# Autodesk Inventor assembly: Left Claw
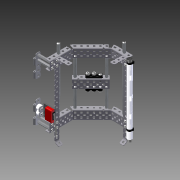
[picture p0: Inventor's stored thumbnail of the model, 180x180]
Saved by Autodesk Inventor 2012 (Build 160160000, 160)
## iProperties
Created: 2011-08-16
Part Number: Left Claw
Document SubType Name: Assembly
Designer: Dakota.Bayer
Author: Dakota.Bayer
## Documents named in this file (26)
- C:\Users\Wade\Documents\1103 Robot - CAD Assembly\Left Claw.iam
- C:\Users\Wade\Documents\1103 Robot - CAD Assembly\2 x 15 bentttttttt.ipt
- C:\Users\Wade\Documents\1103 Robot - CAD Assembly\1 x 20 BENT.ipt
- C:\Users\Wade\Documents\1103 Robot - CAD Assembly\2 x 6 legit.ipt
- C:\Users\Wade\Documents\24C VEX CAD Files\Washers & Spacers\Spacer (Nylon), 0.500''.ipt
- C:\Users\Wade\Documents\24C VEX CAD Files\Standoffs & Couplers\Standoff 2.00''.ipt
- C:\Users\Wade\Documents\24C VEX CAD Files\Other Parts\Shaft Collar (with Set Screw Installed).ipt
- C:\Users\Wade\Documents\24C VEX CAD Files\Other Parts\(Pillow) Bearing Block mod.ipt
- C:\Users\Wade\Documents\24C VEX CAD Files\Washers & Spacers\Spacer (Nylon), 0.250''.ipt
- C:\Users\Wade\Documents\24C VEX CAD Files\Drive Shafts\Drive Shaft (Square Bar) 8''.ipt
- C:\Users\Wade\Documents\1103 Robot - CAD Assembly\VEX-HINGE-2 RevA_1.ipt
- C:\Users\Wade\Documents\1103 Robot - CAD Assembly\Bearing Assembly (end hole).iam
- C:\Users\Wade\Documents\24C VEX CAD Files\Washers & Spacers\Spacer (Nylon), 0.125''.ipt
- C:\Users\Wade\Documents\1103 Robot - CAD Assembly\.375'' Screw & Nylock Nut.iam
- C:\Users\Wade\Documents\24C VEX CAD Files\Standoffs & Couplers\Standoff 5.00''.ipt
- C:\Users\Wade\Documents\24C VEX CAD Files\Screws & Nuts\Screw 8-32 x 0.250''-Silver.ipt
- C:\Users\Wade\Documents\24C VEX CAD Files\Standoffs & Couplers\Standoff 1.50''.ipt
- C:\Users\Wade\Documents\24C VEX CAD Files\Screws & Nuts\Nut 8-32 Nylock.ipt
- C:\Users\Wade\Documents\24C VEX CAD Files\Screws & Nuts\Screw 8-32 x 0.500''-Silver.ipt
- C:\Users\Wade\Documents\24C VEX CAD Files\Standoffs & Couplers\Standoff 1.00''.ipt
- C:\Users\Wade\Documents\24C VEX CAD Files\Motors & Sensors\Limit Switch (Sensor).iam
- C:\Users\Wade\Documents\24C VEX CAD Files\Metal Angles\Short Slotted Angle (Segmented Angle, 1x1x2).ipt
- C:\Users\Wade\Documents\24C VEX CAD Files\Washers & Spacers\Spacer (Nylon), 0.375''.ipt
- C:\Users\Wade\Documents\24C VEX CAD Files\Screws & Nuts\Screw 8-32 x 0.625''-Silver.ipt
- C:\Users\Wade\Documents\24C VEX CAD Files\Washers & Spacers\Spacer (Thin), 4.6mm.ipt
- C:\Users\Wade\Documents\24C VEX CAD Files\Screws & Nuts\Screw 8-32 x 1.750''-Silver.ipt
## Components (93 placed, 25 different names)
1. Standoff 1.50'':1 — Mate:870
2. Standoff 1.50'':2 — Mate:871
3. 2 x 15 bentttttttt:3 — Mate:722, Flush:49, Flush:50, Flush:51, Flush:52, Mate:794, Mate:803, Flush:55, Flush:56, Mate:855, Mate:862, Mate:863, Mate:864, Mate:865, Mate:872, Mate:873, Mate:894, Mate:901, Mate:902, Mate:910, Mate:913, Mate:919, Mate:921
4. Standoff 1.50'':3 — Mate:888, Mate:890
5. Standoff 1.50'':4 — Mate:886, Mate:891
6. 2 x 15 bentttttttt:4 — Mate:796, Mate:797, Mate:804, Mate:805, Mate:806, Flush:57, Mate:851, Mate:879, Mate:881, Mate:883, Mate:885, Mate:892, Mate:893
7. 1 x 20 BENT:3 — Flush:51, Flush:52, Mate:794, Mate:796, Mate:846, Mate:847, Mate:848, Mate:849, Mate:850, Mate:852, Mate:853, Mate:854, Mate:856, Mate:857, Mate:936
8. Standoff 5.00'':1 — Mate:861, Mate:884
9. 2 x 6 legit:2 — Mate:826, Mate:827, Mate:828, Mate:829, Mate:830, Mate:834, Mate:836, Mate:876, Mate:877, Mate:907, Mate:909
10. Standoff 5.00'':2 — Mate:858, Mate:882
11. 1 x 20 BENT:4 — Mate:722, Flush:49, Flush:50, Mate:797, Mate:837, Mate:838, Mate:839, Mate:840, Mate:841, Mate:842, Mate:896, Mate:903
12. Shaft Collar (with Set Screw Installed):1 — Flush:53, Angle:2, Flush:54, Mate:900
13. Shaft Collar (with Set Screw Installed):2 — Mate:815, Flush:54, Flush:58
14. Spacer (Nylon), 0.250'':1 — Mate:808, Mate:809, Mate:810, Mate:811
15. Spacer (Nylon), 0.500'':1 — Mate:808, Mate:809
16. Spacer (Nylon), 0.500'':2 — Mate:810, Mate:811
17. Spacer (Nylon), 0.500'':3
18. Spacer (Nylon), 0.500'':4 — Mate:798, Mate:812, Mate:817
19. Spacer (Nylon), 0.500'':5
20. Spacer (Nylon), 0.500'':6
21. Spacer (Nylon), 0.500'':7
22. Spacer (Nylon), 0.500'':8
23. Spacer (Nylon), 0.500'':9
24. Spacer (Nylon), 0.500'':10
25. Spacer (Nylon), 0.500'':11
26. Spacer (Nylon), 0.500'':12
27. Spacer (Nylon), 0.500'':13 — Mate:798, Mate:813, Mate:814, Mate:815, Mate:818
28. Standoff 2.00'':1 — Mate:859, Mate:874
29. Standoff 2.00'':2 — Mate:860, Mate:875
30. Standoff 2.00'':3 — Mate:880, Mate:906
31. Standoff 2.00'':4 — Mate:878, Mate:908
32. (Pillow) Bearing Block mod:1 — Mate:803, Mate:894, Mate:899, Mate:900, Mate:901, Mate:905
33. (Pillow) Bearing Block mod:2 — Mate:804, Mate:805, Mate:806, Mate:812, Mate:816, Mate:817, Mate:895, Mate:898
34. Spacer (Nylon), 0.250'':2 — Mate:813, Mate:814, Mate:816
35. Drive Shaft (Square Bar) 8'':1 — Mate:818, Flush:53, Angle:2, Flush:58
36. VEX-HINGE-2 RevA_1:1 — Flush:55, Flush:56, Mate:825, Mate:868, Mate:869
37. VEX-HINGE-2 RevA_1:2 — Mate:825, Flush:57, Mate:887, Mate:889, Mate:926, Mate:927, Mate:928, Mate:929, Mate:943, Mate:944
38. Bearing Assembly (end hole):1 [sub-assembly] — Mate:826, Mate:827, Mate:828, Mate:829, Mate:831, Mate:832, Mate:833, Mate:953, Mate:955
39. Bearing Assembly (end hole):2 [sub-assembly] — Mate:830, Mate:831, Mate:832, Mate:835, Mate:956
40. Spacer (Nylon), 0.125'':1 — Mate:833, Mate:834
41. Spacer (Nylon), 0.125'':2 — Mate:835, Mate:836
42. .375'' Screw & Nylock Nut:1 [sub-assembly] — Mate:837, Mate:838, Mate:839
43. .375'' Screw & Nylock Nut:5 [sub-assembly] — Mate:853, Mate:856, Mate:857
44. .375'' Screw & Nylock Nut:7 [sub-assembly] — Mate:840, Mate:841, Mate:842
45. .375'' Screw & Nylock Nut:9 [sub-assembly] — Mate:846, Mate:850, Mate:851
46. .375'' Screw & Nylock Nut:10 [sub-assembly] — Mate:847, Mate:848, Mate:849
47. .375'' Screw & Nylock Nut:12 [sub-assembly] — Mate:852, Mate:854, Mate:855
48. Screw 8-32 x 0.250''-Silver:1 — Mate:859, Mate:864
49. Screw 8-32 x 0.250''-Silver:2 — Mate:858, Mate:865, Mate:911
50. Screw 8-32 x 0.250''-Silver:3 — Mate:860, Mate:863
51. Screw 8-32 x 0.250''-Silver:4 — Mate:861, Mate:862, Mate:912
52. Screw 8-32 x 0.250''-Silver:5 — Mate:868
53. Screw 8-32 x 0.250''-Silver:6 — Mate:869
54. Screw 8-32 x 0.250''-Silver:7 — Mate:870, Mate:872
55. Screw 8-32 x 0.250''-Silver:8 — Mate:871, Mate:873
56. Screw 8-32 x 0.250''-Silver:9 — Mate:875, Mate:877
57. Screw 8-32 x 0.250''-Silver:10 — Mate:874, Mate:876
58. Screw 8-32 x 0.250''-Silver:11 — Mate:880, Mate:881
59. Screw 8-32 x 0.250''-Silver:12 — Mate:878, Mate:879
60. Screw 8-32 x 0.250''-Silver:13 — Mate:882, Mate:883
61. Screw 8-32 x 0.250''-Silver:14 — Mate:884, Mate:885
62. Screw 8-32 x 0.250''-Silver:15 — Mate:888, Mate:889
63. Screw 8-32 x 0.250''-Silver:16 — Mate:886, Mate:887
64. Screw 8-32 x 0.250''-Silver:17 — Mate:891, Mate:893
65. Screw 8-32 x 0.250''-Silver:18 — Mate:890, Mate:892
66. Nut 8-32 Nylock:1 — Mate:897, Mate:898
67. Screw 8-32 x 0.500''-Silver:1 — Mate:895, Mate:896, Mate:897
68. Nut 8-32 Nylock:2 — Mate:904, Mate:905
69. Screw 8-32 x 0.500''-Silver:2 — Mate:899, Mate:902, Mate:903, Mate:904
70. Screw 8-32 x 0.250''-Silver:19 — Mate:906, Mate:907
71. Screw 8-32 x 0.250''-Silver:20 — Mate:908, Mate:909
72. Standoff 1.00'':1 — Mate:910, Mate:911, Mate:914, Mate:915, Mate:920
73. Standoff 1.00'':2 — Mate:912, Mate:913, Mate:916, Mate:917, Mate:918
74. Screw 8-32 x 0.250''-Silver:21 — Mate:914, Mate:915
75. Screw 8-32 x 0.250''-Silver:22 — Mate:916, Mate:917
76. Screw 8-32 x 0.250''-Silver:23 — Mate:920, Mate:921
77. Screw 8-32 x 0.250''-Silver:24 — Mate:918, Mate:919
78. Limit Switch (Sensor):1 [sub-assembly] — Mate:935, Mate:936, Mate:947, Mate:948
79. Screw 8-32 x 0.625''-Silver:3
80. Short Slotted Angle (Segmented Angle, 1x1x2):1 — Mate:922, Mate:923, Mate:924, Mate:925, Mate:932, Mate:933, Mate:934, Mate:939, Mate:951, Mate:952
81. Spacer (Nylon), 0.375'':1 — Mate:922, Mate:924, Mate:926, Mate:929, Mate:937
82. Spacer (Nylon), 0.375'':2 — Mate:923, Mate:925, Mate:927, Mate:928
83. Nut 8-32 Nylock:3 — Mate:950, Mate:951
84. Nut 8-32 Nylock:4 — Mate:942, Mate:944
85. Nut 8-32 Nylock:5 — Mate:943
86. Spacer (Thin), 4.6mm:2 — Mate:934, Mate:945
87. Spacer (Thin), 4.6mm:1 — Mate:932, Mate:933, Mate:935, Mate:946
88. Screw 8-32 x 0.625''-Silver:2 — Mate:937, Mate:939, Mate:942
89. Nut 8-32 Nylock:6 — Mate:949, Mate:952
90. Screw 8-32 x 0.500''-Silver:3 — Mate:946, Mate:948, Mate:949
91. Screw 8-32 x 0.500''-Silver:4 — Mate:945, Mate:947, Mate:950
92. Nut 8-32 Nylock:7 — Mate:954, Mate:956
93. Screw 8-32 x 1.750''-Silver:1 — Mate:953, Mate:954, Mate:955
## Relationships (217: Mate 188, Tangent 18, Flush 10, Angle 1)
- [Mate]: Standoff 1.50'':1 ↔ 2 x 15 bentttttttt:3
- [Tangent] (0.2286 mm): Standoff 1.50'':1 ↔ 2 x 15 bentttttttt:3
- [Tangent] (0.2286 mm): Standoff 1.50'':1 ↔ 2 x 15 bentttttttt:3
- [Tangent] (0.2286 mm): Standoff 1.50'':2 ↔ 2 x 15 bentttttttt:3
- [Mate]: Standoff 1.50'':3 ↔ 2 x 15 bentttttttt:4
- [Tangent] (0.2286 mm): Standoff 1.50'':4 ↔ 2 x 15 bentttttttt:4
- [Tangent] (0.2286 mm): Standoff 1.50'':4 ↔ 2 x 15 bentttttttt:4
- [Tangent] (0.2286 mm): Standoff 1.50'':3 ↔ 2 x 15 bentttttttt:4
- [Mate]: 2 x 15 bentttttttt:3 ↔ Standoff 5.00'':1
- [Tangent] (0.2286 mm): 2 x 15 bentttttttt:3 ↔ Standoff 5.00'':1
- [Tangent] (0.2286 mm): 2 x 15 bentttttttt:3 ↔ Standoff 5.00'':1
- [Mate]: 2 x 15 bentttttttt:3 ↔ Standoff 5.00'':2
- [Tangent] (0.2286 mm): 2 x 15 bentttttttt:3 ↔ Standoff 5.00'':2
- [Tangent] (0.2286 mm): 2 x 15 bentttttttt:3 ↔ Standoff 5.00'':2
- Mate:722: 2 x 15 bentttttttt:3 ↔ 1 x 20 BENT:4
- Flush:49: 2 x 15 bentttttttt:3 ↔ 1 x 20 BENT:4
- Flush:50: 2 x 15 bentttttttt:3 ↔ 1 x 20 BENT:4
- [Mate]: Spacer (Nylon), 0.500'':2 ↔ Spacer (Nylon), 0.500'':3
- [Mate]: Spacer (Nylon), 0.500'':3 ↔ Spacer (Nylon), 0.500'':4
- [Mate]: Spacer (Nylon), 0.500'':2 ↔ Spacer (Nylon), 0.500'':3
- [Mate]: Spacer (Nylon), 0.500'':3 ↔ Spacer (Nylon), 0.500'':4
- [Mate]: Spacer (Nylon), 0.500'':5 ↔ Spacer (Nylon), 0.500'':6
- [Mate]: Spacer (Nylon), 0.500'':5 ↔ Spacer (Nylon), 0.500'':7
- [Mate]: Spacer (Nylon), 0.500'':7 ↔ Spacer (Nylon), 0.500'':8
- [Mate]: Spacer (Nylon), 0.500'':8 ↔ Spacer (Nylon), 0.500'':9
- [Mate]: Spacer (Nylon), 0.500'':9 ↔ Spacer (Nylon), 0.500'':10
- [Mate]: Spacer (Nylon), 0.500'':10 ↔ Spacer (Nylon), 0.500'':11
- [Mate]: Spacer (Nylon), 0.500'':11 ↔ Spacer (Nylon), 0.500'':12
- [Mate]: Spacer (Nylon), 0.500'':5 ↔ Spacer (Nylon), 0.500'':6
- [Mate]: Spacer (Nylon), 0.500'':5 ↔ Spacer (Nylon), 0.500'':7
- [Mate]: Spacer (Nylon), 0.500'':7 ↔ Spacer (Nylon), 0.500'':8
- [Mate]: Spacer (Nylon), 0.500'':8 ↔ Spacer (Nylon), 0.500'':9
- [Mate]: Spacer (Nylon), 0.500'':9 ↔ Spacer (Nylon), 0.500'':10
- [Mate]: Spacer (Nylon), 0.500'':10 ↔ Spacer (Nylon), 0.500'':11
- [Mate]: Spacer (Nylon), 0.500'':11 ↔ Spacer (Nylon), 0.500'':12
- [Mate]: Spacer (Nylon), 0.500'':1 ↔ Spacer (Nylon), 0.500'':12
- [Mate]: Spacer (Nylon), 0.500'':1 ↔ Spacer (Nylon), 0.500'':12
- Flush:51: 2 x 15 bentttttttt:3 ↔ 1 x 20 BENT:3
- Flush:52: 2 x 15 bentttttttt:3 ↔ 1 x 20 BENT:3
- [Mate]: 2 x 6 legit:2 ↔ Standoff 2.00'':1
- [Mate]: 2 x 6 legit:2 ↔ Standoff 2.00'':2
- [Tangent] (0.2286 mm): 2 x 6 legit:2 ↔ Standoff 2.00'':1
- [Tangent] (0.2286 mm): 2 x 6 legit:2 ↔ Standoff 2.00'':1
- [Tangent] (0.2286 mm): 2 x 6 legit:2 ↔ Standoff 2.00'':2
- [Tangent] (0.2286 mm): 2 x 6 legit:2 ↔ Standoff 2.00'':2
- [Mate]: 2 x 15 bentttttttt:3 ↔ Standoff 2.00'':1
- [Tangent] (0.2286 mm): 2 x 15 bentttttttt:3 ↔ Standoff 2.00'':1
- [Tangent] (0.2286 mm): 2 x 15 bentttttttt:3 ↔ Standoff 2.00'':1
- [Tangent] (0.2286 mm): 2 x 15 bentttttttt:3 ↔ Standoff 2.00'':2
- [Tangent] (0.2286 mm): 2 x 15 bentttttttt:3 ↔ Standoff 2.00'':2
- [Mate]: 2 x 6 legit:2 ↔ Standoff 2.00'':3
- [Mate]: 2 x 6 legit:2 ↔ Standoff 2.00'':4
- [Mate]: Standoff 2.00'':2 ↔ Standoff 2.00'':4
- [Mate]: Standoff 2.00'':1 ↔ Standoff 2.00'':3
- Mate:794: 2 x 15 bentttttttt:3 ↔ 1 x 20 BENT:3
- [Mate]: 2 x 15 bentttttttt:4 ↔ Standoff 5.00'':1
- Mate:796: 2 x 15 bentttttttt:4 ↔ 1 x 20 BENT:3
- Mate:797: 2 x 15 bentttttttt:4 ↔ 1 x 20 BENT:4
- Mate:798: Spacer (Nylon), 0.500'':4 ↔ Spacer (Nylon), 0.500'':13
- [Mate]: Shaft Collar (with Set Screw Installed):2 ↔ Spacer (Nylon), 0.500'':13
- [Mate]: Shaft Collar (with Set Screw Installed):1 ↔ Spacer (Nylon), 0.500'':6
- Mate:803 (2.3114 mm): 2 x 15 bentttttttt:3 ↔ (Pillow) Bearing Block mod:1
- Mate:804: 2 x 15 bentttttttt:4 ↔ (Pillow) Bearing Block mod:2
- Mate:805 (2.3114 mm): 2 x 15 bentttttttt:4 ↔ (Pillow) Bearing Block mod:2
- Mate:806 (2.3114 mm): 2 x 15 bentttttttt:4 ↔ (Pillow) Bearing Block mod:2
- Mate:808: Spacer (Nylon), 0.250'':1 ↔ Spacer (Nylon), 0.500'':1
- Mate:809: Spacer (Nylon), 0.250'':1 ↔ Spacer (Nylon), 0.500'':1
- Mate:810: Spacer (Nylon), 0.250'':1 ↔ Spacer (Nylon), 0.500'':2
- Mate:811: Spacer (Nylon), 0.250'':1 ↔ Spacer (Nylon), 0.500'':2
- Mate:812: Spacer (Nylon), 0.500'':4 ↔ (Pillow) Bearing Block mod:2
- Mate:813: Spacer (Nylon), 0.500'':13 ↔ Spacer (Nylon), 0.250'':2
- Mate:814: Spacer (Nylon), 0.500'':13 ↔ Spacer (Nylon), 0.250'':2
- Mate:815: Shaft Collar (with Set Screw Installed):2 ↔ Spacer (Nylon), 0.500'':13
- Mate:816 (3.175 mm): (Pillow) Bearing Block mod:2 ↔ Spacer (Nylon), 0.250'':2
- Mate:817 (3.175 mm): Spacer (Nylon), 0.500'':4 ↔ (Pillow) Bearing Block mod:2
- Mate:818: Spacer (Nylon), 0.500'':13 ↔ Drive Shaft (Square Bar) 8'':1
- Flush:53: Shaft Collar (with Set Screw Installed):1 ↔ Drive Shaft (Square Bar) 8'':1
- Angle:2 (0 deg): Shaft Collar (with Set Screw Installed):1 ↔ Drive Shaft (Square Bar) 8'':1
- Flush:54: Shaft Collar (with Set Screw Installed):1 ↔ Shaft Collar (with Set Screw Installed):2
- [Mate] (2.3114 mm): Standoff 1.50'':2 ↔ 2 x 15 bentttttttt:3
- [Mate]: Standoff 1.50'':2 ↔ 2 x 15 bentttttttt:3
- [Mate]: Standoff 1.50'':2 ↔ VEX-HINGE-2 RevA_1:1
- Flush:55: 2 x 15 bentttttttt:3 ↔ VEX-HINGE-2 RevA_1:1
- Flush:56: 2 x 15 bentttttttt:3 ↔ VEX-HINGE-2 RevA_1:1
- [Mate]: Standoff 1.50'':4 ↔ 2 x 15 bentttttttt:4
- [Mate] (2.3114 mm): Standoff 1.50'':3 ↔ 2 x 15 bentttttttt:4
- [Mate]: Standoff 1.50'':3 ↔ VEX-HINGE-2 RevA_1:2
- Mate:825: VEX-HINGE-2 RevA_1:1 ↔ VEX-HINGE-2 RevA_1:2
- Flush:57: 2 x 15 bentttttttt:4 ↔ VEX-HINGE-2 RevA_1:2
- Mate:826: 2 x 6 legit:2 ↔ Bearing Assembly (end hole):1
- Mate:827 (2.3114 mm): 2 x 6 legit:2 ↔ Bearing Assembly (end hole):1
- Mate:828 (2.3114 mm): 2 x 6 legit:2 ↔ Bearing Assembly (end hole):1
- Mate:829 (2.3114 mm): 2 x 6 legit:2 ↔ Bearing Assembly (end hole):1
- Mate:830: 2 x 6 legit:2 ↔ Bearing Assembly (end hole):2
- Mate:831: Bearing Assembly (end hole):1 ↔ Bearing Assembly (end hole):2
- Mate:832: Bearing Assembly (end hole):1 ↔ Bearing Assembly (end hole):2
- Mate:833: Bearing Assembly (end hole):1 ↔ Spacer (Nylon), 0.125'':1
- Mate:834: 2 x 6 legit:2 ↔ Spacer (Nylon), 0.125'':1
- Mate:835: Bearing Assembly (end hole):2 ↔ Spacer (Nylon), 0.125'':2
- Mate:836: 2 x 6 legit:2 ↔ Spacer (Nylon), 0.125'':2
- Mate:837: 1 x 20 BENT:4 ↔ .375'' Screw & Nylock Nut:1
- Mate:838 (2.3114 mm): 1 x 20 BENT:4 ↔ .375'' Screw & Nylock Nut:1
- Mate:839 (2.3114 mm): 1 x 20 BENT:4 ↔ .375'' Screw & Nylock Nut:1
- Mate:840: 1 x 20 BENT:4 ↔ .375'' Screw & Nylock Nut:7
- Mate:841 (2.3114 mm): 1 x 20 BENT:4 ↔ .375'' Screw & Nylock Nut:7
- Mate:842 (2.3114 mm): 1 x 20 BENT:4 ↔ .375'' Screw & Nylock Nut:7
- Mate:846: 1 x 20 BENT:3 ↔ .375'' Screw & Nylock Nut:9
- Mate:847: 1 x 20 BENT:3 ↔ .375'' Screw & Nylock Nut:10
- Mate:848 (2.3114 mm): 1 x 20 BENT:3 ↔ .375'' Screw & Nylock Nut:10
- Mate:849 (2.3114 mm): 1 x 20 BENT:3 ↔ .375'' Screw & Nylock Nut:10
- Mate:850 (2.3114 mm): 1 x 20 BENT:3 ↔ .375'' Screw & Nylock Nut:9
- Mate:851 (2.3114 mm): 2 x 15 bentttttttt:4 ↔ .375'' Screw & Nylock Nut:9
- Mate:852: 1 x 20 BENT:3 ↔ .375'' Screw & Nylock Nut:12
- Mate:853: 1 x 20 BENT:3 ↔ .375'' Screw & Nylock Nut:5
- Mate:854 (2.3114 mm): 1 x 20 BENT:3 ↔ .375'' Screw & Nylock Nut:12
- Mate:855 (2.3114 mm): 2 x 15 bentttttttt:3 ↔ .375'' Screw & Nylock Nut:12
- Mate:856 (2.3114 mm): 1 x 20 BENT:3 ↔ .375'' Screw & Nylock Nut:5
- Mate:857 (2.3114 mm): 1 x 20 BENT:3 ↔ .375'' Screw & Nylock Nut:5
- Mate:858: Standoff 5.00'':2 ↔ Screw 8-32 x 0.250''-Silver:2
- Mate:859: Standoff 2.00'':1 ↔ Screw 8-32 x 0.250''-Silver:1
- Mate:860: Standoff 2.00'':2 ↔ Screw 8-32 x 0.250''-Silver:3
- Mate:861: Standoff 5.00'':1 ↔ Screw 8-32 x 0.250''-Silver:4
- Mate:862: 2 x 15 bentttttttt:3 ↔ Screw 8-32 x 0.250''-Silver:4
- Mate:863: 2 x 15 bentttttttt:3 ↔ Screw 8-32 x 0.250''-Silver:3
- Mate:864: 2 x 15 bentttttttt:3 ↔ Screw 8-32 x 0.250''-Silver:1
- Mate:865: 2 x 15 bentttttttt:3 ↔ Screw 8-32 x 0.250''-Silver:2
- [Mate]: Standoff 1.50'':2 ↔ Screw 8-32 x 0.250''-Silver:6
- [Mate]: Standoff 1.50'':1 ↔ Screw 8-32 x 0.250''-Silver:5
- Mate:868: VEX-HINGE-2 RevA_1:1 ↔ Screw 8-32 x 0.250''-Silver:5
- Mate:869: VEX-HINGE-2 RevA_1:1 ↔ Screw 8-32 x 0.250''-Silver:6
- Mate:870: Standoff 1.50'':1 ↔ Screw 8-32 x 0.250''-Silver:7
- Mate:871: Standoff 1.50'':2 ↔ Screw 8-32 x 0.250''-Silver:8
- Mate:872: 2 x 15 bentttttttt:3 ↔ Screw 8-32 x 0.250''-Silver:7
- Mate:873: 2 x 15 bentttttttt:3 ↔ Screw 8-32 x 0.250''-Silver:8
- Mate:874: Standoff 2.00'':1 ↔ Screw 8-32 x 0.250''-Silver:10
- Mate:875: Standoff 2.00'':2 ↔ Screw 8-32 x 0.250''-Silver:9
- Mate:876: 2 x 6 legit:2 ↔ Screw 8-32 x 0.250''-Silver:10
- Mate:877: 2 x 6 legit:2 ↔ Screw 8-32 x 0.250''-Silver:9
- Mate:878: Standoff 2.00'':4 ↔ Screw 8-32 x 0.250''-Silver:12
- Mate:879: 2 x 15 bentttttttt:4 ↔ Screw 8-32 x 0.250''-Silver:12
- Mate:880: Standoff 2.00'':3 ↔ Screw 8-32 x 0.250''-Silver:11
- Mate:881: 2 x 15 bentttttttt:4 ↔ Screw 8-32 x 0.250''-Silver:11
- Mate:882: Standoff 5.00'':2 ↔ Screw 8-32 x 0.250''-Silver:13
- Mate:883: 2 x 15 bentttttttt:4 ↔ Screw 8-32 x 0.250''-Silver:13
- Mate:884: Standoff 5.00'':1 ↔ Screw 8-32 x 0.250''-Silver:14
- Mate:885: 2 x 15 bentttttttt:4 ↔ Screw 8-32 x 0.250''-Silver:14
- Mate:886: Standoff 1.50'':4 ↔ Screw 8-32 x 0.250''-Silver:16
- Mate:887: VEX-HINGE-2 RevA_1:2 ↔ Screw 8-32 x 0.250''-Silver:16
- Mate:888: Standoff 1.50'':3 ↔ Screw 8-32 x 0.250''-Silver:15
- Mate:889: VEX-HINGE-2 RevA_1:2 ↔ Screw 8-32 x 0.250''-Silver:15
- Mate:890: Standoff 1.50'':3 ↔ Screw 8-32 x 0.250''-Silver:18
- Mate:891: Standoff 1.50'':4 ↔ Screw 8-32 x 0.250''-Silver:17
- Mate:892: 2 x 15 bentttttttt:4 ↔ Screw 8-32 x 0.250''-Silver:18
- Mate:893: 2 x 15 bentttttttt:4 ↔ Screw 8-32 x 0.250''-Silver:17
- Mate:894: 2 x 15 bentttttttt:3 ↔ (Pillow) Bearing Block mod:1
- Mate:895: (Pillow) Bearing Block mod:2 ↔ Screw 8-32 x 0.500''-Silver:1
- Mate:896: 1 x 20 BENT:4 ↔ Screw 8-32 x 0.500''-Silver:1
- Mate:897: Nut 8-32 Nylock:1 ↔ Screw 8-32 x 0.500''-Silver:1
- Mate:898: (Pillow) Bearing Block mod:2 ↔ Nut 8-32 Nylock:1
- Mate:899: (Pillow) Bearing Block mod:1 ↔ Screw 8-32 x 0.500''-Silver:2
- Mate:900: Shaft Collar (with Set Screw Installed):1 ↔ (Pillow) Bearing Block mod:1
- Mate:901: 2 x 15 bentttttttt:3 ↔ (Pillow) Bearing Block mod:1
- Mate:902 (2.3114 mm): 2 x 15 bentttttttt:3 ↔ Screw 8-32 x 0.500''-Silver:2
- Flush:58: Shaft Collar (with Set Screw Installed):2 ↔ Drive Shaft (Square Bar) 8'':1
- Mate:903: 1 x 20 BENT:4 ↔ Screw 8-32 x 0.500''-Silver:2
- Mate:904: Nut 8-32 Nylock:2 ↔ Screw 8-32 x 0.500''-Silver:2
- Mate:905: (Pillow) Bearing Block mod:1 ↔ Nut 8-32 Nylock:2
- Mate:906: Standoff 2.00'':3 ↔ Screw 8-32 x 0.250''-Silver:19
- Mate:907: 2 x 6 legit:2 ↔ Screw 8-32 x 0.250''-Silver:19
- Mate:908: Standoff 2.00'':4 ↔ Screw 8-32 x 0.250''-Silver:20
- Mate:909: 2 x 6 legit:2 ↔ Screw 8-32 x 0.250''-Silver:20
- Mate:910: 2 x 15 bentttttttt:3 ↔ Standoff 1.00'':1
- Mate:911: Screw 8-32 x 0.250''-Silver:2 ↔ Standoff 1.00'':1
- Mate:912: Screw 8-32 x 0.250''-Silver:4 ↔ Standoff 1.00'':2
- Mate:913: 2 x 15 bentttttttt:3 ↔ Standoff 1.00'':2
- Mate:914: Standoff 1.00'':1 ↔ Screw 8-32 x 0.250''-Silver:21
- Mate:915: Standoff 1.00'':1 ↔ Screw 8-32 x 0.250''-Silver:21
- Mate:916: Standoff 1.00'':2 ↔ Screw 8-32 x 0.250''-Silver:22
- Mate:917: Standoff 1.00'':2 ↔ Screw 8-32 x 0.250''-Silver:22
- Mate:918: Standoff 1.00'':2 ↔ Screw 8-32 x 0.250''-Silver:24
- Mate:919: 2 x 15 bentttttttt:3 ↔ Screw 8-32 x 0.250''-Silver:24
- Mate:920: Standoff 1.00'':1 ↔ Screw 8-32 x 0.250''-Silver:23
- Mate:921: 2 x 15 bentttttttt:3 ↔ Screw 8-32 x 0.250''-Silver:23
- Mate:922: Short Slotted Angle (Segmented Angle, 1x1x2):1 ↔ Spacer (Nylon), 0.375'':1
- Mate:923: Short Slotted Angle (Segmented Angle, 1x1x2):1 ↔ Spacer (Nylon), 0.375'':2
- Mate:924: Short Slotted Angle (Segmented Angle, 1x1x2):1 ↔ Spacer (Nylon), 0.375'':1
- Mate:925: Short Slotted Angle (Segmented Angle, 1x1x2):1 ↔ Spacer (Nylon), 0.375'':2
- Mate:926: VEX-HINGE-2 RevA_1:2 ↔ Spacer (Nylon), 0.375'':1
- Mate:927 (2.3114 mm): VEX-HINGE-2 RevA_1:2 ↔ Spacer (Nylon), 0.375'':2
- Mate:928 (2.3114 mm): VEX-HINGE-2 RevA_1:2 ↔ Spacer (Nylon), 0.375'':2
- Mate:929 (2.3114 mm): VEX-HINGE-2 RevA_1:2 ↔ Spacer (Nylon), 0.375'':1
- [Mate]: Short Slotted Angle (Segmented Angle, 1x1x2):1 ↔ Spacer (Thin), 4.6mm:2
- Mate:932: Short Slotted Angle (Segmented Angle, 1x1x2):1 ↔ Spacer (Thin), 4.6mm:1
- Mate:933: Short Slotted Angle (Segmented Angle, 1x1x2):1 ↔ Spacer (Thin), 4.6mm:1
- Mate:934: Short Slotted Angle (Segmented Angle, 1x1x2):1 ↔ Spacer (Thin), 4.6mm:2
- Mate:935: Limit Switch (Sensor):1 ↔ Spacer (Thin), 4.6mm:1
- Mate:936: 1 x 20 BENT:3 ↔ Limit Switch (Sensor):1
- Mate:937: Spacer (Nylon), 0.375'':1 ↔ Screw 8-32 x 0.625''-Silver:2
- [Mate]: Screw 8-32 x 0.625''-Silver:3 ↔ Spacer (Nylon), 0.375'':2
- Mate:939: Short Slotted Angle (Segmented Angle, 1x1x2):1 ↔ Screw 8-32 x 0.625''-Silver:2
- [Mate]: Screw 8-32 x 0.625''-Silver:3 ↔ Short Slotted Angle (Segmented Angle, 1x1x2):1
- [Mate]: Screw 8-32 x 0.625''-Silver:3 ↔ Nut 8-32 Nylock:5
- Mate:942: Nut 8-32 Nylock:4 ↔ Screw 8-32 x 0.625''-Silver:2
- Mate:943: VEX-HINGE-2 RevA_1:2 ↔ Nut 8-32 Nylock:5
- Mate:944: VEX-HINGE-2 RevA_1:2 ↔ Nut 8-32 Nylock:4
- Mate:945: Spacer (Thin), 4.6mm:2 ↔ Screw 8-32 x 0.500''-Silver:4
- Mate:946: Spacer (Thin), 4.6mm:1 ↔ Screw 8-32 x 0.500''-Silver:3
- Mate:947: Limit Switch (Sensor):1 ↔ Screw 8-32 x 0.500''-Silver:4
- Mate:948: Limit Switch (Sensor):1 ↔ Screw 8-32 x 0.500''-Silver:3
- Mate:949: Nut 8-32 Nylock:6 ↔ Screw 8-32 x 0.500''-Silver:3
- Mate:950: Nut 8-32 Nylock:3 ↔ Screw 8-32 x 0.500''-Silver:4
- Mate:951: Short Slotted Angle (Segmented Angle, 1x1x2):1 ↔ Nut 8-32 Nylock:3
- Mate:952: Short Slotted Angle (Segmented Angle, 1x1x2):1 ↔ Nut 8-32 Nylock:6
- Mate:953: Bearing Assembly (end hole):1 ↔ Screw 8-32 x 1.750''-Silver:1
- Mate:954: Nut 8-32 Nylock:7 ↔ Screw 8-32 x 1.750''-Silver:1
- Mate:955: Bearing Assembly (end hole):1 ↔ Screw 8-32 x 1.750''-Silver:1
- Mate:956: Bearing Assembly (end hole):2 ↔ Nut 8-32 Nylock:7
